# Autodesk Inventor assembly: wheel_with_mounts
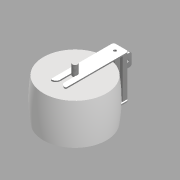
[picture p0: Inventor's stored thumbnail of the model, 180x180]
Saved by Autodesk Inventor 2021.3 (Build 253353000, 353)
## iProperties
Created: 2021-05-27
Part Number: wheel_with_mounts
Document SubType Name: Assembly
Designer: gisen
Author: gisen
## Documents named in this file (5)
- C:\Users\gisen\workspace\beetle_inventor_model\suspension\wheel_with_mounts.iam
- C:\Users\gisen\workspace\beetle_inventor_model\suspension\6inch_wheel.ipt
- C:\Users\gisen\workspace\beetle_inventor_model\suspension\CAM\wheel_mount.ipt
- C:\Users\gisen\workspace\beetle_inventor_model\suspension\CAM\wheel_frame_mount.ipt
- C:\Users\gisen\workspace\beetle_inventor_model\suspension\frame\AFS-3030-97.ipt
## Components (5 placed, 4 different names)
1. 6inch_wheel:1 — メイト:1, メイト:2, メイト:3, フラッシュ:3, フラッシュ:10, メイト:12
2. wheel_mount — メイト:3, フラッシュ:3, フラッシュ:10, フラッシュ:12, メイト:12, フラッシュ:13, メイト:14, メイト:15, フラッシュ:14
3. wheel_mount:2 — メイト:13, メイト:16, フラッシュ:14, メイト:18
4. AFS-3030-97:1 — フラッシュ:13, メイト:13, メイト:14, メイト:15, メイト:16, メイト:17, フラッシュ:15
5. wheel_frame_mount:1 — メイト:17, フラッシュ:15, メイト:18
## Relationships (16: Mate 10, Flush 6)
- メイト:1 [Mate]: 6inch_wheel:1
- メイト:2 [Mate]: 6inch_wheel:1
- メイト:3 [Mate]: 6inch_wheel:1 ↔ wheel_mount
- フラッシュ:3 [Flush]: 6inch_wheel:1 ↔ wheel_mount
- フラッシュ:10 [Flush]: 6inch_wheel:1 ↔ wheel_mount
- フラッシュ:12 [Flush]: wheel_mount
- メイト:12 [Mate]: 6inch_wheel:1 ↔ wheel_mount
- フラッシュ:13 [Flush]: wheel_mount ↔ AFS-3030-97:1
- メイト:13 [Mate]: wheel_mount:2 ↔ AFS-3030-97:1
- メイト:14 [Mate]: wheel_mount ↔ AFS-3030-97:1
- メイト:15 [Mate]: wheel_mount ↔ AFS-3030-97:1
- メイト:16 [Mate]: wheel_mount:2 ↔ AFS-3030-97:1
- フラッシュ:14 [Flush]: wheel_mount ↔ wheel_mount:2
- メイト:17 [Mate]: AFS-3030-97:1 ↔ wheel_frame_mount:1
- フラッシュ:15 [Flush]: AFS-3030-97:1 ↔ wheel_frame_mount:1
- メイト:18 [Mate]: wheel_mount:2 ↔ wheel_frame_mount:1
